# Autodesk Inventor assembly: J005779
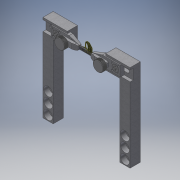
[picture p0: Inventor's stored thumbnail of the model, 180x180]
Saved by Autodesk Inventor 2018.2 (Build 222227000, 227)
## iProperties
Created: 2016-08-08
Vendor: HHMI: JRC - ID&F
Document SubType Name: Assembly
Designer: ARNOLDJ
Part Number: J005779
Description: HEAD POST AND MOUNTING BARS
RuleStatus: InUse
AfterDocSave0: file://Part Number Cleaner
DESIGN DEPARTMENT: HHMI: JRC - ID&F
ALTERED ITEM PART NUMBER: N/A
ALTERED ITEM VENDOR: N/A
ALTERED ITEM DESCRIPTION: N/A
Revision Number: 0
## Documents named in this file (11)
- C:\_WORKSPACE\DATA\PROJECTS\VARIOUS HEADPOST DESIGNS FOR MULTIPLE LABS\MCAD\HEAD POST AND MOUNTING BARS.iam
- C:\_WORKSPACE\DATA\PROJECTS\VARIOUS HEADPOST DESIGNS FOR MULTIPLE LABS\MCAD\BarrelCtxPlateSlopedLeft.ipt
- C:\_WORKSPACE\DATA\PROJECTS\VARIOUS HEADPOST DESIGNS FOR MULTIPLE LABS\MCAD\HeadPostHolderBottom.ipt
- C:\_WORKSPACE\DATA\PROJECTS\VARIOUS HEADPOST DESIGNS FOR MULTIPLE LABS\MCAD\HeadPostHolderTop.ipt
- C:\_WORKSPACE\DATA\PROJECTS\VARIOUS HEADPOST DESIGNS FOR MULTIPLE LABS\MCAD\HEAD MOUNT ARM ML.ipt
- C:\_WORKSPACE\DATA\PROJECTS\VARIOUS HEADPOST DESIGNS FOR MULTIPLE LABS\MCAD\HEAD MOUNT ARM MR.ipt
- C:\_WORKSPACE\DATA\PROJECTS\VARIOUS HEADPOST DESIGNS FOR MULTIPLE LABS\MCAD\91771A197.ipt
- C:\_WORKSPACE\DATA\PROJECTS\VARIOUS HEADPOST DESIGNS FOR MULTIPLE LABS\MCAD\92141A009.ipt
- C:\_WORKSPACE\DATA\PROJECTS\VARIOUS HEADPOST DESIGNS FOR MULTIPLE LABS\MCAD\91185A440.ipt
- C:\_WORKSPACE\DATA\PROJECTS\VARIOUS HEADPOST DESIGNS FOR MULTIPLE LABS\MCAD\91841A009.ipt
- C:\_WORKSPACE\DATA\PROJECTS\VARIOUS HEADPOST DESIGNS FOR MULTIPLE LABS\MCAD\KS style headpost with three epoxy holes.ipt
## Components (16 placed, 10 different names)
1. BarrelCtxPlateSlopedLeft:1 — Mate:1, Mate:2, Mate:3, Mate:4, Mate:5, Mate:6, Flush:5
2. HeadPostHolderBottom:1 — Mate:1, Mate:2, Mate:3, Mate:9, Mate:10, Mate:13, Mate:14, Flush:2, Flush:3, Mate:15, Mate:29
3. HeadPostHolderBottom:2 — Mate:4, Mate:5, Mate:6, Mate:7, Mate:8, Mate:11, Mate:12, Flush:1, Flush:4, Mate:16
4. HeadPostHolderTop:1 — Mate:7, Mate:8, Mate:23, Mate:24
5. HeadPostHolderTop:2 — Mate:9, Mate:10, Mate:21, Mate:22
6. HEAD MOUNT ARM ML:1 — Mate:11, Mate:12, Flush:1, Mate:19
7. HEAD MOUNT ARM MR:1 — Mate:13, Mate:14, Flush:2, Mate:17
8. 91771A197:1 — Flush:3, Mate:15, Mate:18, Mate:26
9. 91771A197:2 — Flush:4, Mate:16, Mate:20, Mate:28
10. 92141A009:1 — Mate:17, Mate:18, Mate:25
11. 92141A009:2 — Mate:19, Mate:20, Mate:27
12. 91185A440:1 — Mate:23, Mate:24
13. 91185A440:2 — Mate:21, Mate:22
14. 91841A009:1 — Mate:25, Mate:26
15. 91841A009:2 — Mate:27, Mate:28
16. KS style headpost with three epoxy holes:1 — Flush:5, Mate:29
## Relationships (34: Mate 29, Flush 5)
- Mate:1: BarrelCtxPlateSlopedLeft:1 ↔ HeadPostHolderBottom:1
- Mate:2: BarrelCtxPlateSlopedLeft:1 ↔ HeadPostHolderBottom:1
- Mate:3: BarrelCtxPlateSlopedLeft:1 ↔ HeadPostHolderBottom:1
- Mate:4: BarrelCtxPlateSlopedLeft:1 ↔ HeadPostHolderBottom:2
- Mate:5: BarrelCtxPlateSlopedLeft:1 ↔ HeadPostHolderBottom:2
- Mate:6: BarrelCtxPlateSlopedLeft:1 ↔ HeadPostHolderBottom:2
- Mate:7: HeadPostHolderBottom:2 ↔ HeadPostHolderTop:1
- Mate:8: HeadPostHolderBottom:2 ↔ HeadPostHolderTop:1
- Mate:9: HeadPostHolderBottom:1 ↔ HeadPostHolderTop:2
- Mate:10: HeadPostHolderBottom:1 ↔ HeadPostHolderTop:2
- Mate:11: HeadPostHolderBottom:2 ↔ HEAD MOUNT ARM ML:1
- Mate:12: HeadPostHolderBottom:2 ↔ HEAD MOUNT ARM ML:1
- Flush:1 (11.049 mm): HeadPostHolderBottom:2 ↔ HEAD MOUNT ARM ML:1
- Mate:13: HeadPostHolderBottom:1 ↔ HEAD MOUNT ARM MR:1
- Mate:14: HeadPostHolderBottom:1 ↔ HEAD MOUNT ARM MR:1
- Flush:2 (11.049 mm): HeadPostHolderBottom:1 ↔ HEAD MOUNT ARM MR:1
- Flush:3: HeadPostHolderBottom:1 ↔ 91771A197:1
- Mate:15: HeadPostHolderBottom:1 ↔ 91771A197:1
- Flush:4: HeadPostHolderBottom:2 ↔ 91771A197:2
- Mate:16: HeadPostHolderBottom:2 ↔ 91771A197:2
- Mate:17: HEAD MOUNT ARM MR:1 ↔ 92141A009:1
- Mate:18: 91771A197:1 ↔ 92141A009:1
- Mate:19: HEAD MOUNT ARM ML:1 ↔ 92141A009:2
- Mate:20: 91771A197:2 ↔ 92141A009:2
- Mate:21: HeadPostHolderTop:2 ↔ 91185A440:2
- Mate:22: HeadPostHolderTop:2 ↔ 91185A440:2
- Mate:23: HeadPostHolderTop:1 ↔ 91185A440:1
- Mate:24: HeadPostHolderTop:1 ↔ 91185A440:1
- Mate:25: 92141A009:1 ↔ 91841A009:1
- Mate:26: 91771A197:1 ↔ 91841A009:1
- Mate:27: 92141A009:2 ↔ 91841A009:2
- Mate:28: 91771A197:2 ↔ 91841A009:2
- Flush:5: BarrelCtxPlateSlopedLeft:1 ↔ KS style headpost with three epoxy holes:1
- Mate:29: HeadPostHolderBottom:1 ↔ KS style headpost with three epoxy holes:1
